# Autodesk Inventor assembly: TestAssem
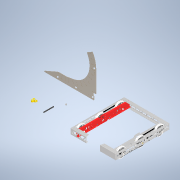
[picture p0: Inventor's stored thumbnail of the model, 180x180]
Saved by Autodesk Inventor 2020 (Build 240168000, 168)
## iProperties
Created: 2020-11-25
Part Number: TestAssem
Document SubType Name: Assembly
Designer: srini
Author: srini
## Documents named in this file (6)
- C:\Users\srini\Documents\FRC\2020\TestAssem.iam
- C:\Users\srini\Documents\FRC\2020\thriftybearingmount.ipt
- C:\Users\srini\Documents\FRC\2020\DriveBase2020.iam
- C:\Users\srini\Documents\FRC\2020\IntakeShooter\OutsideCLarge.ipt
- C:\Users\srini\Documents\FRC\2020\ThunderHex_6in.ipt
- C:\Users\srini\Documents\FRC\2020\TTB-0004_TheThriftyBushing.ipt
## Components (6 placed, 5 different names)
1. thriftybearingmount:1 — Insert:1
2. DriveBase2020:1 [sub-assembly]
3. OutsideCLarge:1
4. ThunderHex_6in:1
5. TTB-0004_TheThriftyBushing:1 — Insert:1
6. TTB-0004_TheThriftyBushing:2
## Relationships (1: Insert 1)
- Insert:1: thriftybearingmount:1 ↔ TTB-0004_TheThriftyBushing:1
